# Autodesk Inventor assembly: ベルト
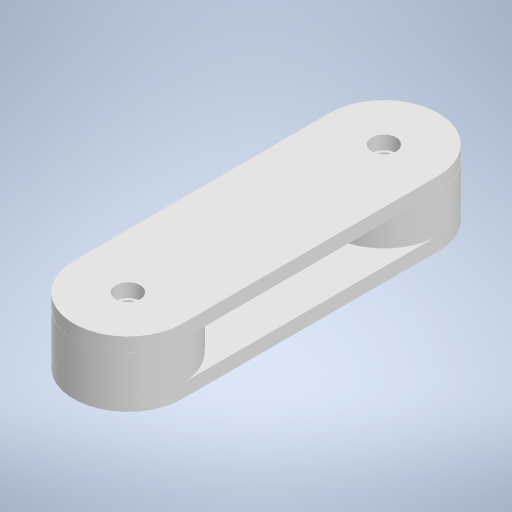
[picture p0: Inventor's stored thumbnail of the model, 512x512]
Saved by Autodesk Inventor 2024.1 (Build 281209000, 209)
## iProperties
Created: 2024-03-26
Part Number: ベルト
Document SubType Name: Assembly
Designer: hibik
Author: hibik
## Documents named in this file (3)
- C:\Users\hibik\Desktop\ロボメカ\2年\新歓\ベルトコンベア\ベルト.iam
- C:\Users\hibik\Desktop\ロボメカ\2年\新歓\ベルトコンベア\ベルト.ipt
- C:\Users\hibik\Desktop\ロボメカ\2年\新歓\ベルトコンベア\ベルト_支柱.ipt
## Components (4 placed, 2 different names)
1. ベルト:1 — 挿入:1, 挿入:2
2. ベルト:2 — 挿入:3, 挿入:4
3. ベルト_支柱:1 — 挿入:1, 挿入:4
4. ベルト_支柱:2 — 挿入:2, 挿入:3
## Relationships (4: Insert 4)
- 挿入:1 [Insert]: ベルト:1 ↔ ベルト_支柱:1
- 挿入:2 [Insert]: ベルト:1 ↔ ベルト_支柱:2
- 挿入:3 [Insert]: ベルト:2 ↔ ベルト_支柱:2
- 挿入:4 [Insert]: ベルト:2 ↔ ベルト_支柱:1
